# Autodesk Inventor assembly: 头洞四方轴套
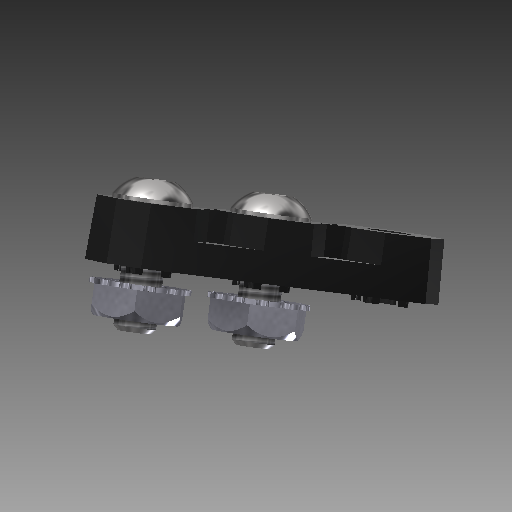
[picture p0: Inventor's stored thumbnail of the model, 512x512]
Saved by Autodesk Inventor 2019.3 (Build 233278000, 278)
## iProperties
Created: 2018-09-04
Part Number: 头洞四方轴套
Material: 常规
Document SubType Name: Assembly
Designer: aresp
Mass: 6.09763 g
Surface Area: 27.9754 cm^2
Volume: 2.17078 cm^3
Density: 2.80895 g/cm^3
d8: 0.000 mm
d9: 0.000 mm
d13: 0.000 mm
d2: 0.000 mm
Author: aresp
## Documents named in this file (4)
- D:\cad\工作空间\头洞四方轴套.iam
- D:\cad\零件库\Bearing Flat.ipt
- D:\cad\零件库\螺丝螺帽\Screw 8-32 x 0.500'' - Black.ipt
- D:\cad\零件库\螺丝螺帽\Nut 8-32 Keps.ipt
## Components (5 placed, 3 different names)
1. Bearing Flat:1
2. Screw 8-32 x 0.500'' - Black:1
3. Screw 8-32 x 0.500'' - Black:2
4. Nut 8-32 Keps:1
5. Nut 8-32 Keps:2
## Relationships (2: Insert 2)
- [Insert]: Bearing Flat:1 ↔ Screw 8-32 x 0.500'' - Black:1
- [Insert]: Bearing Flat:1 ↔ Screw 8-32 x 0.500'' - Black:2
